# Autodesk Inventor assembly: ARM001
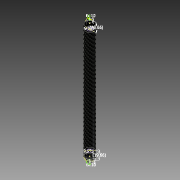
[picture p0: Inventor's stored thumbnail of the model, 180x180]
Saved by Autodesk Inventor 2015 SP1 (Build 190203100, 203)
## iProperties
Created: 2015-05-12
Part Number: ARM001
Document SubType Name: Assembly
Designer: rhornbak
Author: rhornbak
## Documents named in this file (3)
- Z:\Delta Robot\Mechanical\ARM001.iam
- Z:\Delta Robot\Mechanical\ROD001 - Rod 20x18mm.ipt
- Z:\Delta Robot\Mechanical\ROD002 - Rod End 20x18mm.ipt
## Components (3 placed, 2 different names)
1. ROD001 - Rod 20x18mm:1 — Mate:3, Mate:4
2. ROD002 - Rod End 20x18mm:1 — Mate:3
3. ROD002 - Rod End 20x18mm:2 — Mate:4
## Relationships (2: Mate 2)
- Mate:3: ROD001 - Rod 20x18mm:1 ↔ ROD002 - Rod End 20x18mm:1
- Mate:4: ROD001 - Rod 20x18mm:1 ↔ ROD002 - Rod End 20x18mm:2
